# Autodesk Inventor assembly: mount_hcsr04
Saved by Autodesk Inventor 2021 (Build 250183000, 183)
## iProperties
Created: 2021-01-20
Part Number: mount_hcsr04
Document SubType Name: Assembly
Designer: User
Author: User
## Documents named in this file (3)
- D:\SynologyDrive\tcodev\tco-cad\mount_hcsr04\mount_hcsr04.iam
- D:\SynologyDrive\tcodev\tco-cad\common\hcsr04\hcsr04.iam
- D:\SynologyDrive\tcodev\tco-cad\mount_hcsr04\mount.ipt
## Components (2 placed, 2 different names)
1. hcsr04:1 [sub-assembly] — Flush:1
2. mount:1 — Flush:1
## Relationships (1: Flush 1)
- Flush:1: hcsr04:1 ↔ mount:1
